# Autodesk Inventor assembly: axis_4_top_frame_motor_iam
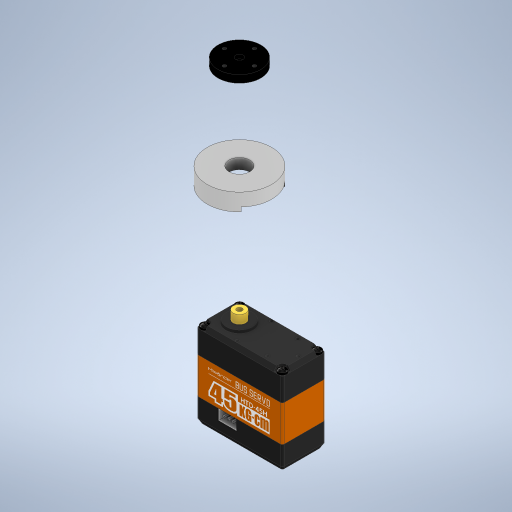
[picture p0: Inventor's stored thumbnail of the model, 512x512]
Saved by Autodesk Inventor 2024.1 (Build 281209000, 209)
## iProperties
Created: 2023-10-28
Part Number: axis_4_top_frame_motor_iam
Document SubType Name: Assembly
Designer: chanh
Author: chanh
## Documents named in this file (4)
- C:\Users\chanh\OneDrive - 연세대학교 (Yonsei University)\로봇\Humanoid\Roboin Humanoid Project\Inventor\rh_plus_7_axis_robot_arm_hardware\Part\Frame\gripper\axis_4_top_frame_motor_iam.iam
- C:\Users\chanh\OneDrive - 연세대학교 (Yonsei University)\로봇\Humanoid\Roboin Humanoid Project\Inventor\rh_plus_7_axis_robot_arm_hardware\Part\HTD-45H, Horn\HTD-45H\HTD-45H.iam
- C:\Users\chanh\OneDrive - 연세대학교 (Yonsei University)\로봇\Humanoid\Roboin Humanoid Project\Inventor\rh_plus_7_axis_robot_arm_hardware\Part\Frame\axis_4_top_frame2.ipt
- C:\Users\chanh\OneDrive - 연세대학교 (Yonsei University)\로봇\Humanoid\Roboin Humanoid Project\Inventor\rh_plus_7_axis_robot_arm_hardware\Part\HTD-45H, Horn\Horn\Top Horn.ipt
## Components (3 placed, 3 different names)
1. HTD-45H:1 [sub-assembly] — Flush:1, Flush:2, Flush:3, Mate:1, Flush:4, Mate:2, Rotational:1
2. axis_4_top_frame2:1 — Mate:1, Flush:4, Mate:2
3. Top Horn:1 — Rotational:1
## Relationships (7: Flush 4, Mate 2, RevoluteJoint 1)
- Flush:1: HTD-45H:1
- Flush:2: HTD-45H:1
- Flush:3: HTD-45H:1
- Mate:1 (50 mm): HTD-45H:1 ↔ axis_4_top_frame2:1
- Flush:4: HTD-45H:1 ↔ axis_4_top_frame2:1
- Mate:2: HTD-45H:1 ↔ axis_4_top_frame2:1
- Rotational:1 [RevoluteJoint] (100 mm): HTD-45H:1 ↔ Top Horn:1
